# Autodesk Inventor assembly: PWTR-0091
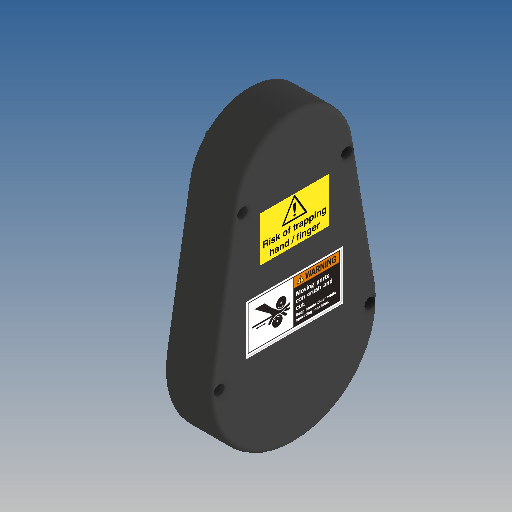
[picture p0: Inventor's stored thumbnail of the model, 512x512]
Saved by Autodesk Inventor 2021.1 (Build 251245000, 245)
## iProperties
Created: 2020-08-28
Part Number: PWTR-0091
Document SubType Name: Assembly
Designer: alid
Description: Honda GX160 Drive Unit
Author: alid
Revision Number: A
## Documents named in this file (12)
- C:\Vault Workspace\Design Data\Projects\PRJ0095\PWTR-Components\PWTR-0091.iam
- C:\Vault Workspace\Design Data\Projects\PRJ0095\PWTR-Components\PWTR-0084.ipt
- C:\Vault Workspace\Design Data\Projects\PRJ0095\PWTR-Components\PWTR-0090.ipt
- C:\Vault Workspace\Design Data\Projects\PRJ0095\PWTR-Components\PWTR-0092.ipt
- C:\Vault Workspace\Design Data\Projects\PRJ0095\PWTR-Components\PWTR-0093.ipt
- C:\Vault Workspace\Design Data\Projects\PRJ0095\PWTR-Components\PWTR-0094.ipt
- C:\Vault Workspace\Design Data\Projects\PRJ0095\PWTR-Components\PWTR-0097.ipt
- C:\Vault Workspace\Design Data\Projects\PRJ0095\PWTR-Components\PWTR-0096.ipt
- C:\Vault Workspace\Design Data\Projects\PRJ0095\PWTR-Components\PWTR-0115.ipt
- C:\Vault Workspace\Design Data\Projects\PRJ0095\PWTR-Components\PWTR-0116.ipt
- C:\Vault Workspace\Design Data\Projects\PRJ0095\PWTR-Components\PWTR-0125.ipt
- C:\Vault Workspace\Design Data\Projects\PRJ0095\PWTR-Components\PWTR-0126.ipt
## Components (25 placed, 11 different names)
1. Backing Plate — Rigid:1, Insert:1, Insert:2, Insert:3, Insert:4, Angle:1, Insert:14, Insert:15, Insert:16, Insert:17, Insert:18
2. Cover — Rigid:1, Insert:5, Insert:6, Insert:7, Insert:8, Mate:1
3. PWTR-0126:1 — Insert:1
4. PWTR-0092:2 — Insert:3
5. PWTR-0092:3 — Insert:2
6. PWTR-0092:4 — Insert:4
7. PWTR-0093:1 — Insert:5
8. PWTR-0093:2 — Insert:7
9. PWTR-0093:3 — Insert:6
10. PWTR-0093:4 — Insert:8
11. PWTR-0096:1 — Insert:10, Insert:11, Flush:1
12. Coupling — Insert:13, Mate:1, Flush:1
13. PWTR-0115:1 — Insert:11, Insert:12
14. PWTR-0116:1 — Insert:12
15. PWTR-0116:2 — Insert:13
16. PWTR-0125:1 — Insert:14
17. PWTR-0126:3 — Insert:15
18. PWTR-0125:2 — Insert:16
19. PWTR-0126:2 — Insert:17
20. PWTR-0097:1 — Insert:10, Angle:1
21. PWTR-0097:2
22. PWTR-0125:3 — Insert:18
23. PWTR-0125:4
24. PWTR-0125:5
25. PWTR-0125:6
## Component patterns: (2 elements, first: PWTR-0097:1), (4 elements, first: PWTR-0125:3)
## Relationships (22: Insert 18, WeldJoint 1, Mate 1, Flush 1, Angle 1)
- Rigid:1 [WeldJoint] (-3 mm): Backing Plate ↔ Cover
- Insert:1: Backing Plate ↔ PWTR-0126:1
- Insert:2: Backing Plate ↔ PWTR-0092:3
- Insert:3: Backing Plate ↔ PWTR-0092:2
- Insert:4: Backing Plate ↔ PWTR-0092:4
- Insert:5: Cover ↔ PWTR-0093:1
- Insert:6: Cover ↔ PWTR-0093:3
- Insert:7: Cover ↔ PWTR-0093:2
- Insert:8: Cover ↔ PWTR-0093:4
- [Insert] (2 mm): Backing Plate ↔ PWTR-0096:1
- Insert:10: PWTR-0096:1 ↔ PWTR-0097:1
- Insert:11: PWTR-0096:1 ↔ PWTR-0115:1
- Insert:12: PWTR-0115:1 ↔ PWTR-0116:1
- Insert:13: Coupling ↔ PWTR-0116:2
- Mate:1: Cover ↔ Coupling
- Flush:1: PWTR-0096:1 ↔ Coupling
- Angle:1 (180 deg): Backing Plate ↔ PWTR-0097:1
- Insert:14: Backing Plate ↔ PWTR-0125:1
- Insert:15 (5 mm): Backing Plate ↔ PWTR-0126:3
- Insert:16: Backing Plate ↔ PWTR-0125:2
- Insert:17 (5 mm): Backing Plate ↔ PWTR-0126:2
- Insert:18: Backing Plate ↔ PWTR-0125:3
